# Autodesk Inventor assembly: fem2
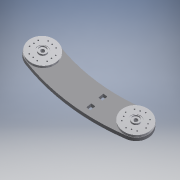
[picture p0: Inventor's stored thumbnail of the model, 180x180]
Saved by Autodesk Inventor 2019 (Build 230136000, 136)
## iProperties
Created: 2023-04-17
Part Number: fem2
Document SubType Name: Assembly
Designer: Analuam
Author: Analuam
## Documents named in this file (3)
- D:\Dek Diyah\fem2.iam
- D:\Dek Diyah\fem.ipt
- D:\Dek Diyah\servomg996r\Acople circular.ipt
## Components (3 placed, 2 different names)
1. fem:1 — Insert:1, Insert:2
2. Acople circular:1 — Insert:1
3. Acople circular:2 — Insert:2
## Relationships (2: Insert 2)
- Insert:1: fem:1 ↔ Acople circular:1
- Insert:2: fem:1 ↔ Acople circular:2
